# Autodesk Inventor assembly: Palme
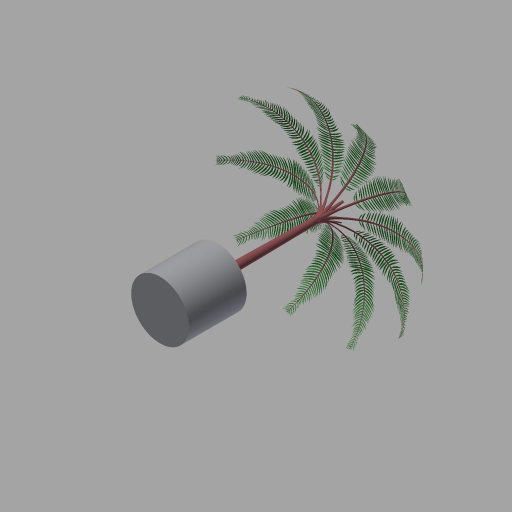
[picture p0: Inventor's stored thumbnail of the model, 512x512]
Saved by Autodesk Inventor 2023.2 (Build 272271000, 271)
## iProperties
Created: 2023-02-01
Part Number: Palme
Material: Generisch
Document SubType Name: Assembly
Designer: Raoul Messerli
Author: Raoul Messerli
## Documents named in this file (3)
- E:\GitHub\Pflanzenwagen\20_Inventor\10_Vorlage\Palme.iam
- E:\GitHub\Pflanzenwagen\20_Inventor\10_Vorlage\Topf.ipt
- E:\GitHub\Pflanzenwagen\20_Inventor\10_Vorlage\tree.ipt
## Components (2 placed, 2 different names)
1. Topf:1 — Passend:1, Passend:2
2. tree:1 — Passend:1, Passend:2
## Relationships (2: Mate 2)
- Passend:1 [Mate]: Topf:1 ↔ tree:1
- Passend:2 [Mate]: Topf:1 ↔ tree:1
